# Autodesk Inventor assembly: workbench
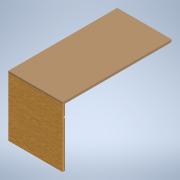
[picture p0: Inventor's stored thumbnail of the model, 180x180]
Saved by Autodesk Inventor 2022 (Build 260153000, 153)
## iProperties
Created: 2022-02-21
Part Number: workbench
Document SubType Name: Assembly
Designer: MarkP
Author: MarkP
## Documents named in this file (4)
- C:\Users\MarkP\Documents\Mark\final\workbench.iam
- C:\Users\MarkP\Documents\Mark\final\desk.ipt
- C:\Users\MarkP\Documents\Mark\final\wallL1.ipt
- C:\Users\MarkP\Documents\Mark\final\wallL2.ipt
## Components (3 placed, 3 different names)
1. desk:1 — Mate:2, Flush:3, Mate:3
2. wallL1:1 — Flush:1, Mate:1, Flush:2, Flush:3
3. wallL2:1 — Flush:1, Mate:1, Flush:2, Mate:2, Mate:3
## Relationships (6: Flush 3, Mate 3)
- Flush:1: wallL1:1 ↔ wallL2:1
- Mate:1: wallL1:1 ↔ wallL2:1
- Flush:2: wallL1:1 ↔ wallL2:1
- Mate:2: desk:1 ↔ wallL2:1
- Flush:3: desk:1 ↔ wallL1:1
- Mate:3: desk:1 ↔ wallL2:1
